# Autodesk Inventor assembly: Gears_Trial
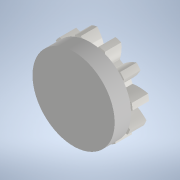
[picture p0: Inventor's stored thumbnail of the model, 180x180]
Saved by Autodesk Inventor 2022 (Build 260153000, 153)
## iProperties
Created: 2022-02-11
Part Number: Gears_Trial
Document SubType Name: Assembly
Designer: Mlees
Author: Mlees
## Documents named in this file (3)
- C:\Users\Mlees\Desktop\504Engineering\Stepper-Servo_Based_Robotic_Arm\Designs\Version_6\Created_Parts\Gears_Trial.iam
- C:\Users\Mlees\Desktop\504Engineering\Stepper-Servo_Based_Robotic_Arm\Designs\Version_6\Created_Parts\Part2.ipt
- C:\Users\Mlees\Desktop\504Engineering\Stepper-Servo_Based_Robotic_Arm\Designs\Version_6\Created_Parts\Gears_Trial\Design Accelerator\Spur Gears1.iam
## Components (2 placed, 2 different names)
1. Part2:1 — Mate:1, Mate:2
2. Spur Gears:1 [sub-assembly] — Mate:1, Mate:2
## Relationships (2: Mate 2)
- Mate:1: Part2:1 ↔ Spur Gears:1
- Mate:2: Part2:1 ↔ Spur Gears:1
